# Autodesk Inventor assembly: A Idler
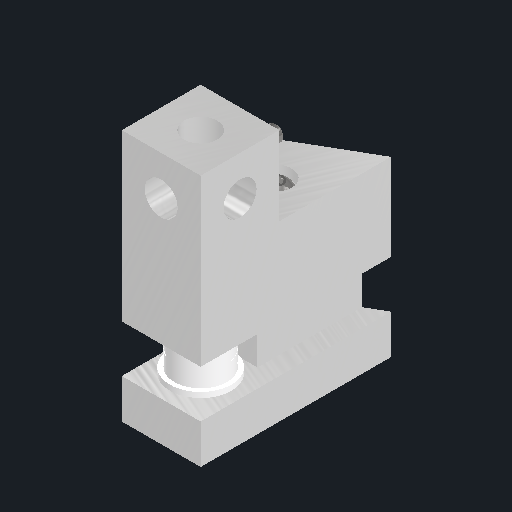
[picture p0: Inventor's stored thumbnail of the model, 512x512]
Saved by Autodesk Inventor 2025.1 (Build 291241020, 241B)
## iProperties
Created: 2025-05-09
Part Number: A Idler
Document SubType Name: Assembly
Designer: AdminForWorker
Title: A Idler
Author: AdminForWorker
## Documents named in this file (3)
- C:\Users\Joshua Eah\Documents\Voron 0.2\CAD\Master Assembly\A Idler.iam
- C:\Users\Joshua Eah\Documents\Voron 0.2\CAD\Master Assembly\Hardware\Hardware Assemblies\Hardware (9).iam
- C:\Users\Joshua Eah\Documents\Voron 0.2\CAD\Machined Parts\Idlers\A Idler\A Idler.ipt
## Components (2 placed, 2 different names)
1. Hardware (9):1 [sub-assembly] — Insert:1
2. A Idler:1 — Insert:1
## Relationships (1: Insert 1)
- Insert:1: Hardware (9):1 ↔ A Idler:1
